# Autodesk Inventor assembly: Top_Assy
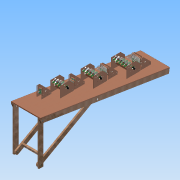
[picture p0: Inventor's stored thumbnail of the model, 180x180]
Saved by Autodesk Inventor 2018.1 (Build 221171000, 171)
## iProperties
Created: 2019-03-18
Part Number: Top_Assy
Document SubType Name: Assembly
Designer: James
Author: James
## Documents named in this file (12)
- C:\Users\admin\Desktop\Ball-Machine\Top Level\Top_Assy.iam
- C:\Users\admin\Desktop\Ball-Machine\Selection Sort\Selection_Assy.iam
- C:\Users\admin\Desktop\Ball-Machine\Pancake Sort\Pancake_Assy.iam
- C:\Users\admin\Desktop\Ball-Machine\Selection Sort\Selection - 4 Lanes\Selection_Assy 4 Lanes.iam
- C:\Users\admin\Desktop\Ball-Machine\Top Level\Top_Slider Assy.iam
- C:\Users\admin\Desktop\Ball-Machine\Selection Sort\Selection - 3 Lanes\Selection_Assy 3 Lanes.iam
- C:\Users\admin\Desktop\Ball-Machine\Selection Sort\Selection - 2 Lanes\Selection_Assy 2 Lanes.iam
- C:\Users\admin\Desktop\Ball-Machine\Pancake Sort\Pancake - 3 Lanes\Pancake_Assy_3 Lanes.iam
- C:\Users\admin\Desktop\Ball-Machine\Pancake Sort\Pancake - 4 Lanes\Pancake_Assy_4 Lanes.iam
- C:\Users\admin\Desktop\Ball-Machine\Top Level\Top_Slider Assy_3 Lanes.iam
- C:\Users\admin\Desktop\Ball-Machine\Top Level\Top_Slider Assy_4 Lanes.iam
- C:\Users\admin\Desktop\Ball-Machine\Top Level\Top_Backboard Assy.iam
## Components (11 placed, 11 different names)
1. Selection_Assy:1 [sub-assembly] — Flush:1, Flush:2, Flush:3, Flush:4, Flush:5, Mate:1, Tangent:1, Tangent:2, Flush:6, Mate:2, Flush:8, Flush:20
2. Pancake_Assy:1 [sub-assembly] — Flush:4, Flush:6, Mate:2, Flush:7, Flush:15, Mate:8
3. Selection_Assy 4 Lanes:1 [sub-assembly] — Flush:5, Flush:8, Flush:9, Flush:11, Mate:3, Flush:12, Flush:15, Mate:5, Mate:6, Tangent:3, Tangent:4, Flush:18, Mate:8
4. Top_Slider Assy:1 [sub-assembly] — Mate:1, Tangent:1, Tangent:2, Flush:7
5. Selection_Assy 3 Lanes:1 [sub-assembly] — Flush:9, Flush:10, Flush:13, Mate:4, Flush:14, Flush:16, Mate:7, Tangent:5, Tangent:6, Flush:19, Mate:9
6. Selection_Assy 2 Lanes:1 [sub-assembly] — Flush:10, Flush:17, Mate:10
7. Pancake_Assy_3 Lanes:1 [sub-assembly] — Flush:13, Mate:4, Flush:14, Flush:17, Mate:10
8. Pancake_Assy_4 Lanes:1 [sub-assembly] — Flush:11, Mate:3, Flush:12, Flush:16, Mate:9
9. Top_Slider Assy_3 Lanes:1 [sub-assembly] — Mate:7, Tangent:5, Tangent:6, Flush:19
10. Top_Slider Assy_4 Lanes:1 [sub-assembly] — Mate:5, Mate:6, Tangent:3, Tangent:4, Flush:18
11. Top_Backboard Assy:1 [sub-assembly] — Angle:1, Flush:20
## Relationships (37: Flush 20, Mate 10, Tangent 6, Angle 1)
- Flush:1: Selection_Assy:1
- Flush:2: Selection_Assy:1
- Flush:3: Selection_Assy:1
- Flush:4 (107.5 mm): Selection_Assy:1 ↔ Pancake_Assy:1
- Flush:5: Selection_Assy:1 ↔ Selection_Assy 4 Lanes:1
- Mate:1 (2 mm): Selection_Assy:1 ↔ Top_Slider Assy:1
- Tangent:1: Selection_Assy:1 ↔ Top_Slider Assy:1
- Tangent:2: Selection_Assy:1 ↔ Top_Slider Assy:1
- Flush:6: Selection_Assy:1 ↔ Pancake_Assy:1
- Mate:2 (160 mm): Selection_Assy:1 ↔ Pancake_Assy:1
- Flush:7: Pancake_Assy:1 ↔ Top_Slider Assy:1
- Flush:8: Selection_Assy:1 ↔ Selection_Assy 4 Lanes:1
- Flush:9: Selection_Assy 4 Lanes:1 ↔ Selection_Assy 3 Lanes:1
- Flush:10: Selection_Assy 3 Lanes:1 ↔ Selection_Assy 2 Lanes:1
- Flush:11: Selection_Assy 4 Lanes:1 ↔ Pancake_Assy_4 Lanes:1
- Mate:3 (160 mm): Selection_Assy 4 Lanes:1 ↔ Pancake_Assy_4 Lanes:1
- Flush:12 (62.5 mm): Selection_Assy 4 Lanes:1 ↔ Pancake_Assy_4 Lanes:1
- Flush:13 (17.5 mm): Selection_Assy 3 Lanes:1 ↔ Pancake_Assy_3 Lanes:1
- Mate:4 (160 mm): Selection_Assy 3 Lanes:1 ↔ Pancake_Assy_3 Lanes:1
- Flush:14: Selection_Assy 3 Lanes:1 ↔ Pancake_Assy_3 Lanes:1
- Flush:15 (150 mm): Pancake_Assy:1 ↔ Selection_Assy 4 Lanes:1
- Flush:16 (150 mm): Selection_Assy 3 Lanes:1 ↔ Pancake_Assy_4 Lanes:1
- Flush:17 (150 mm): Selection_Assy 2 Lanes:1 ↔ Pancake_Assy_3 Lanes:1
- Mate:5 (2 mm): Selection_Assy 4 Lanes:1 ↔ Top_Slider Assy_4 Lanes:1
- Mate:6 (2 mm): Selection_Assy 4 Lanes:1 ↔ Top_Slider Assy_4 Lanes:1
- Tangent:3: Selection_Assy 4 Lanes:1 ↔ Top_Slider Assy_4 Lanes:1
- Tangent:4: Selection_Assy 4 Lanes:1 ↔ Top_Slider Assy_4 Lanes:1
- Flush:18: Selection_Assy 4 Lanes:1 ↔ Top_Slider Assy_4 Lanes:1
- Mate:7 (2 mm): Selection_Assy 3 Lanes:1 ↔ Top_Slider Assy_3 Lanes:1
- Tangent:5: Selection_Assy 3 Lanes:1 ↔ Top_Slider Assy_3 Lanes:1
- Tangent:6: Selection_Assy 3 Lanes:1 ↔ Top_Slider Assy_3 Lanes:1
- Flush:19: Selection_Assy 3 Lanes:1 ↔ Top_Slider Assy_3 Lanes:1
- Mate:8 (160 mm): Pancake_Assy:1 ↔ Selection_Assy 4 Lanes:1
- Mate:9 (160 mm): Selection_Assy 3 Lanes:1 ↔ Pancake_Assy_4 Lanes:1
- Mate:10 (160 mm): Selection_Assy 2 Lanes:1 ↔ Pancake_Assy_3 Lanes:1
- Angle:1 (0 deg): Top_Backboard Assy:1
- Flush:20 (-500 mm): Selection_Assy:1 ↔ Top_Backboard Assy:1
